# Autodesk Inventor assembly: Assembly
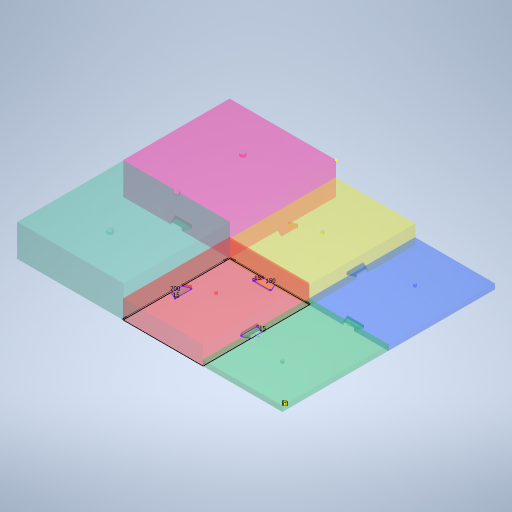
[picture p0: Inventor's stored thumbnail of the model, 512x512]
Saved by Autodesk Inventor 2024 (Build 280153000, 153)
## iProperties
Created: 2024-03-01
Part Number: Assembly
Document SubType Name: Assembly
Designer: laura
Author: laura
## Documents named in this file (7)
- C:\Uni\Semesterprojekt 2\Assembly.iam
- C:\Uni\Semesterprojekt 2\Area nh.ipt
- C:\Uni\Semesterprojekt 2\Area nv.ipt
- C:\Uni\Semesterprojekt 2\Area mh.ipt
- C:\Uni\Semesterprojekt 2\Area mv.ipt
- C:\Uni\Semesterprojekt 2\Area øh1.ipt
- C:\Uni\Semesterprojekt 2\Area øv1.ipt
## Components (6 placed, 6 different names)
1. Area nh:1 — Slider:1, Slider:2
2. Area nv:1 — Slider:1
3. Area mh:1 — Slider:2, Slider:4
4. Area mv:1 — Slider:5
5. Area øh1:1 — Slider:4
6. Area øv1:1 — Slider:5
## Relationships (4: TranslationJoint 4)
- Slider:1 [TranslationJoint]: Area nh:1 ↔ Area nv:1
- Slider:2 [TranslationJoint]: Area nh:1 ↔ Area mh:1
- Slider:4 [TranslationJoint]: Area mh:1 ↔ Area øh1:1
- Slider:5 [TranslationJoint]: Area mv:1 ↔ Area øv1:1
